# Autodesk Inventor assembly: 組合2
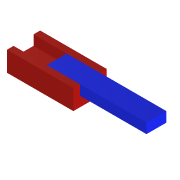
[picture p0: Inventor's stored thumbnail of the model, 180x180]
Saved by Autodesk Inventor 2022 (Build 260153000, 153)
## iProperties
Created: 2023-04-19
Part Number: 組合2
Document SubType Name: Assembly
Designer: JOU
Author: JOU
## Documents named in this file (3)
- C:\Users\JOU\Desktop\git\Special-project\ppt用\組合2.iam
- C:\Users\JOU\Desktop\git\Special-project\ppt用\零件2.ipt
- C:\Users\JOU\Desktop\git\Special-project\ppt用\零件3.ipt
## Components (2 placed, 2 different names)
1. 零件2:1 — 貼合:1, 貼合:2, 齊平:1
2. 零件3:1 — 貼合:1, 貼合:2, 齊平:1
## Relationships (3: Mate 2, Flush 1)
- 貼合:1 [Mate]: 零件2:1 ↔ 零件3:1
- 貼合:2 [Mate]: 零件2:1 ↔ 零件3:1
- 齊平:1 [Flush] (-20 mm): 零件2:1 ↔ 零件3:1
